# Autodesk Inventor assembly: Rotor
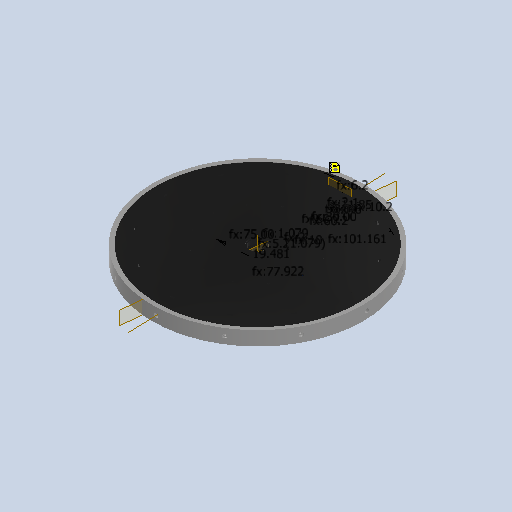
[picture p0: Inventor's stored thumbnail of the model, 512x512]
Saved by Autodesk Inventor 2022.2 (Build 262287000, 287)
## iProperties
Created: 2022-07-21
Part Number: Rotor
Document SubType Name: Assembly
Designer: ABL
Author: ABL
## Documents named in this file (9)
- C:\GitHubRepos\PHYS-12-Website\content\portfolio\Final Project\CAD\Axial Flux Motor iProject\Rotor.iam
- C:\GitHubRepos\PHYS-12-Website\content\portfolio\Final Project\CAD\Axial Flux Motor iProject\RotorBody.ipt
- C:\GitHubRepos\PHYS-12-Website\content\portfolio\Final Project\CAD\Axial Flux Motor iProject\DriveMagnet.ipt
- C:\GitHubRepos\PHYS-12-Website\content\portfolio\Final Project\CAD\Axial Flux Motor iProject\HalbachMagnet.ipt
- C:\GitHubRepos\PHYS-12-Website\content\portfolio\Final Project\CAD\Axial Flux Motor iProject\SensorMagnet.ipt
- C:\GitHubRepos\PHYS-12-Website\content\portfolio\Final Project\CAD\Axial Flux Motor iProject\SensorMagnet_Reverse.ipt
- C:\GitHubRepos\PHYS-12-Website\content\portfolio\Final Project\CAD\Axial Flux Motor iProject\DriveMagnet_Reverse.ipt
- C:\GitHubRepos\PHYS-12-Website\content\portfolio\Final Project\CAD\Axial Flux Motor iProject\HalbachMagnet_MIR1.ipt
- C:\GitHubRepos\PHYS-12-Website\content\portfolio\Final Project\CAD\Axial Flux Motor iProject\MotorGlobalParameters.xlsx
## Components (61 placed, 7 different names)
1. RotorBody:1 — Mate:1, Mate:2, Mate:3, Mate:4, Flush:7, Mate:5, Mate:7, Mate:8, Mate:9, Angle:1, Mate:10, Mate:11, Mate:12, Mate:13, Mate:14, Mate:15, Mate:16, Flush:8
2. SensorMagnet:1 — Mate:7, Mate:8
3. SensorMagnet:2
4. SensorMagnet:3
5. SensorMagnet:4
6. SensorMagnet:5
7. SensorMagnet:6
8. SensorMagnet_Reverse:1 — Mate:10, Mate:11
9. SensorMagnet_Reverse:2
10. SensorMagnet_Reverse:3
11. SensorMagnet_Reverse:4
12. SensorMagnet_Reverse:5
13. SensorMagnet_Reverse:6
14. DriveMagnet:1 — Mate:1, Mate:2, Mate:3
15. DriveMagnet:2
16. HalbachMagnet:1 — Mate:4, Flush:7, Mate:5
17. HalbachMagnet:2
18. DriveMagnet:3
19. DriveMagnet:4
20. HalbachMagnet:3
21. HalbachMagnet:4
22. DriveMagnet:5
23. DriveMagnet:6
24. HalbachMagnet:5
25. HalbachMagnet:6
26. DriveMagnet:7
27. DriveMagnet:8
28. HalbachMagnet:7
29. HalbachMagnet:8
30. DriveMagnet:9
31. DriveMagnet:10
32. HalbachMagnet:9
33. HalbachMagnet:10
34. DriveMagnet:11
35. DriveMagnet:12
36. HalbachMagnet:11
37. HalbachMagnet:12
38. DriveMagnet_Reverse:1 — Mate:12, Mate:13, Mate:14
39. DriveMagnet_Reverse:2
40. HalbachMagnet_MIR1:1
41. HalbachMagnet_MIR1:2 — Mate:15, Mate:16, Flush:8
42. DriveMagnet_Reverse:3
43. DriveMagnet_Reverse:4
44. HalbachMagnet_MIR1:3
45. HalbachMagnet_MIR1:4
46. DriveMagnet_Reverse:5
47. DriveMagnet_Reverse:6
48. HalbachMagnet_MIR1:5
49. HalbachMagnet_MIR1:6
50. DriveMagnet_Reverse:7
51. DriveMagnet_Reverse:8
52. HalbachMagnet_MIR1:7
53. HalbachMagnet_MIR1:8
54. DriveMagnet_Reverse:9
55. DriveMagnet_Reverse:10
56. HalbachMagnet_MIR1:9
57. HalbachMagnet_MIR1:10
58. DriveMagnet_Reverse:11
59. DriveMagnet_Reverse:12
60. HalbachMagnet_MIR1:11
61. HalbachMagnet_MIR1:12
## Component patterns: NorthMagnets (6 elements), SouthMagnets (6 elements), DriveMagnetStack (2 elements), HalbachMagnetStack (2 elements), DriveMagnetStack:2 (2 elements), HalbachMagnetStack:2 (2 elements), DriveMagnetStack:3 (2 elements), HalbachMagnetStack:3 (2 elements), DriveMagnetStack:4 (2 elements), HalbachMagnetStack:4 (2 elements), DriveMagnetStack:5 (2 elements), HalbachMagnetStack:5 (2 elements), DriveMagnetStack:6 (2 elements), HalbachMagnetStack:6 (2 elements), DriveMagnetStack_Reverse (2 elements), HalbachMagnetStack_Reverse (2 elements), (2 elements, first: DriveMagnet_Reverse:3), (2 elements, first: HalbachMagnet_MIR1:3), (2 elements, first: DriveMagnet_Reverse:5), (2 elements, first: HalbachMagnet_MIR1:5), (2 elements, first: DriveMagnet_Reverse:7), (2 elements, first: HalbachMagnet_MIR1:7), (2 elements, first: DriveMagnet_Reverse:9), (2 elements, first: HalbachMagnet_MIR1:9), (2 elements, first: DriveMagnet_Reverse:11), (2 elements, first: HalbachMagnet_MIR1:11)
## Relationships (18: Mate 15, Flush 2, Angle 1)
- Mate:1: RotorBody:1 ↔ DriveMagnet:1
- Mate:2 (0.1 mm): RotorBody:1 ↔ DriveMagnet:1
- Mate:3 (0.1 mm): RotorBody:1 ↔ DriveMagnet:1
- Mate:4 (0.1 mm): RotorBody:1 ↔ HalbachMagnet:1
- Flush:7 (0.1 mm): RotorBody:1 ↔ HalbachMagnet:1
- Mate:5: RotorBody:1 ↔ HalbachMagnet:1
- Mate:7: RotorBody:1 ↔ SensorMagnet:1
- Mate:8: RotorBody:1 ↔ SensorMagnet:1
- Mate:9: RotorBody:1
- Angle:1 (90 deg): RotorBody:1
- Mate:10: RotorBody:1 ↔ SensorMagnet_Reverse:1
- Mate:11: RotorBody:1 ↔ SensorMagnet_Reverse:1
- Mate:12: RotorBody:1 ↔ DriveMagnet_Reverse:1
- Mate:13 (0.1 mm): RotorBody:1 ↔ DriveMagnet_Reverse:1
- Mate:14 (0.1 mm): RotorBody:1 ↔ DriveMagnet_Reverse:1
- Mate:15 (0.1 mm): RotorBody:1 ↔ HalbachMagnet_MIR1:2
- Mate:16: RotorBody:1 ↔ HalbachMagnet_MIR1:2
- Flush:8 (0.1 mm): RotorBody:1 ↔ HalbachMagnet_MIR1:2
## Named parameters: gap = 0.1 mm, airgap = 0.4 mm, driveMagnet_length = 60 mm, driveMagnet_width = 10 mm, driveMagnet_height = 5 mm, halbachMagnet_length = 60 mm, halbachMagnet_width = 10 mm, halbachMagnet_height = 3 mm, sensorMagnet_diameter = 5 mm, sensorMagnet_height = 2.66667 mm, numMagnetSets = 12, numElectromagnets = 9, wallgap = 2 mm, halbachMagnet_numStacked = 2, driveMagnet_centerSpacingRadius = 38.96113 mm, motorRadius = 103.16113 mm, rotorThickness = 14.1 mm, driveMagnet_numStacked = 2, shaftDiameter = 8 mm, flangeBearing_outerDiameter = 16 mm, flangeBearing_innerDiameter = 8 mm, flangeBearing_height = 5 mm, flangeBearing_flangeHeight = 1 mm, flangeBearing_flangeDiameter = 18 mm, magnetTrapNut_height = 1.2 mm, magnetTrapNut_sideToSide = 4 mm, magnetTrapBolt_headHeight = 2 mm, magnetTrapBolt_headDiameter = 3.98 mm, magnetTrapBolt_diameter = 2 mm, statorThickness = 16 mm, rotor_mountingLipHeight = 8 mm, magnetTrapBolt_shaftLength = 20 mm, magnetTrapHexNut_sideToSide = 4 mm, magnetTrapSquareNut_sideLength = 4 mm, magnetTrapSquareNut_height = 1.2 mm, magnetTrapHexNut_height = 1.2 mm, magnetTrap_wingDegrees = 4.443207 deg, magnetTrap_wingOuterDegrees = 11.764706 deg, rotorRadius = 101.16113 mm, rotorBandSquareNut_sideLength = 4 mm, rotorBandHexNut_height = 1.2 mm, rotorBandBolt_shaftLength = 20 mm, rotorBandHexNut_sideToSide = 4 mm, rotorBandSquareNut_height = 1.2 mm, rotorBandBolt_headHeight = 2 mm, rotorBandBolt_headDiameter = 3.98 mm, rotorBandBolt_diameter = 2 mm, rotorBandThickness = 4.1 mm, shaftLength = 200 mm, flangeCoupling_collarOuterDiameter = 16 mm, flangeCoupling_flangeHoleEdgeToEdge = 2.05 mm, flangeCoupling_innerDiameter = 8 mm, flangeCoupling_flangeHoleDiameter = 3.9 mm, flangeCoupling_flangeHeight = 3.1 mm, flangeCoupling_collarHeight = 10 mm, flangeCoupling_flangeDiameter = 32 mm, flangeCoupling_height = 13.1 mm, flangeCoupling_mountHoleDiameter = 3.9 mm, flangeCoupling_mountHoleEdgeToEdge = 2.05 mm, statorRadius = 99.16113 mm, coilThickness = 12 mm, statorMountBolt_diameter = 4 mm, statorMountBolt_headDiameter = 7 mm, statorMountBolt_headHeight = 4 mm, statorMountBolt_shaftLength = 17.1 mm, statorMountHexNut_height = 4 mm, statorMountHexNut_sideToSide = 8 mm, sensorMagnet_ringRadius = 23.48057 mm, coil_percentCoverage = 0.6, statorSpokeDegrees = 4 deg, coil_bulge = 3 mm, coil_cornerRadius = 10 mm, coil_width = 10 mm, statorCoilBolt_shaftLength = 12 mm, statorCoilHexNut_height = 1.2 mm, statorCoilBolt_headHeight = 2 mm, statorCoilBolt_diameter = 2 mm, statorCoilBolt_headDiameter = 3.98 mm, statorCoilHexNut_sideToSide = 4 mm, magnetWire_gauge = 20, magnetWire_outerDiameter = 0.8128 mm, printingLayerHeight = 0.2 mm, circuitBoard_height = 1.6 mm, hallEffectSensor_width = 1.6 mm, hallEffectSensor_length = 3 mm, hallEffectSensor_height = 1.1 mm, hallEffectSensor_pinLength = 0.6 mm, circuitboardMountHexNut_height = 1.2 mm, circuitboardMountHexNut_sideToSide = 4 mm, circuitboardMountBolt_headHeight = 2 mm, circuitboardMountBolt_shaftLength = 12 mm, circuitboardMountBolt_diameter = 2 mm, circuitboardMountBolt_headDiameter = 3.98 mm, statorShellBolt_headDiameter = 5.68 mm, statorShellHexNut_height = 2.3 mm, statorShellBolt_shaftLength = 12.6 mm, statorShellBolt_headHeight = 3 mm, statorShellHexNut_sideToSide = 5.3 mm, statorShellBolt_diameter = 3 mm, statorShellBolt_countersinkDepth = 3.4 mm
